# Autodesk Inventor assembly: Assembly
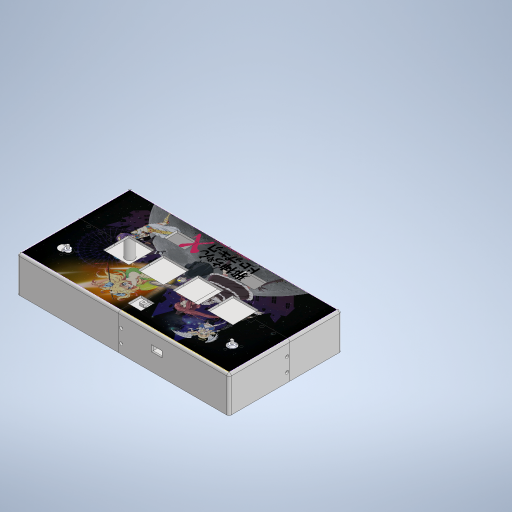
[picture p0: Inventor's stored thumbnail of the model, 512x512]
Saved by Autodesk Inventor 2023 (Build 270158000, 158)
## iProperties
Created: 2024-05-21
Part Number: Assembly
Document SubType Name: Assembly
Designer: Nitrene.P.L
Author: Nitrene.P.L
## Documents named in this file (12)
- E:\Github\AgSDVX\Hardware\Case_new\Assembly.iam
- E:\Github\AgSDVX\Hardware\Case_new\top_A.ipt
- E:\Github\AgSDVX\Hardware\Case_new\top_B.ipt
- E:\Github\AgSDVX\Hardware\Case_new\top_C.ipt
- E:\Github\AgSDVX\Hardware\Case_new\top_D.ipt
- E:\Github\AgSDVX\Hardware\Case\rotary_encoder.ipt
- E:\Github\AgSDVX\Hardware\Case_new\底板_A.ipt
- E:\Github\AgSDVX\Hardware\Case_new\底板_B.ipt
- E:\Github\AgSDVX\Hardware\Case_new\底板_C.ipt
- E:\Github\AgSDVX\Hardware\Case_new\底板_D.ipt
- E:\Github\AgSDVX\Hardware\Case_new\connect.ipt
- E:\Github\AgSDVX\Hardware\Case_new\adder.ipt
## Components (16 placed, 11 different names)
1. top_A:1 — 表面齐平:1, 配合:1, 配合:2, 表面齐平:2, 配合:3, 表面齐平:3, 插入:1, 表面齐平:7, 配合:4, 配合:5, 插入:3
2. top_B:1 — 表面齐平:1, 配合:1, 配合:2, 表面齐平:5, 插入:2, 表面齐平:8, 配合:6, 配合:7, 插入:4
3. top_C:1 — 表面齐平:2, 配合:3, 表面齐平:3, 表面齐平:4, 表面齐平:6, 表面齐平:9, 表面齐平:10, 配合:10, 配合:11
4. top_D:1 — 表面齐平:4, 表面齐平:5, 表面齐平:6, 配合:8, 配合:9
5. rotary_encoder:1 — 插入:1
6. rotary_encoder:2 — 插入:2
7. 底板_A:1 — 表面齐平:8, 配合:6, 配合:7
8. 底板_B:1 — 表面齐平:7, 配合:4, 配合:5
9. 底板_C:1 — 表面齐平:9, 配合:8, 配合:9, 配合:12, 配合:13
10. 底板_D:1 — 表面齐平:10, 配合:10, 配合:11, 配合:14, 配合:15
11. connect:1 — 配合:12
12. connect:2 — 配合:13
13. connect:3 — 配合:14
14. connect:4 — 配合:15
15. adder:1 — 插入:4
16. adder:2 — 插入:3
## Relationships (29: Mate 15, Flush 10, Insert 4)
- 表面齐平:1 [Flush]: top_A:1 ↔ top_B:1
- 配合:1 [Mate]: top_A:1 ↔ top_B:1
- 配合:2 [Mate]: top_A:1 ↔ top_B:1
- 表面齐平:2 [Flush]: top_A:1 ↔ top_C:1
- 配合:3 [Mate]: top_A:1 ↔ top_C:1
- 表面齐平:3 [Flush]: top_A:1 ↔ top_C:1
- 表面齐平:4 [Flush]: top_C:1 ↔ top_D:1
- 表面齐平:5 [Flush]: top_B:1 ↔ top_D:1
- 表面齐平:6 [Flush]: top_C:1 ↔ top_D:1
- 插入:1 [Insert]: top_A:1 ↔ rotary_encoder:1
- 插入:2 [Insert]: top_B:1 ↔ rotary_encoder:2
- 表面齐平:7 [Flush]: top_A:1 ↔ 底板_B:1
- 配合:4 [Mate]: top_A:1 ↔ 底板_B:1
- 配合:5 [Mate]: top_A:1 ↔ 底板_B:1
- 表面齐平:8 [Flush]: top_B:1 ↔ 底板_A:1
- 配合:6 [Mate]: top_B:1 ↔ 底板_A:1
- 配合:7 [Mate]: top_B:1 ↔ 底板_A:1
- 表面齐平:9 [Flush]: top_C:1 ↔ 底板_C:1
- 配合:8 [Mate]: top_D:1 ↔ 底板_C:1
- 配合:9 [Mate]: top_D:1 ↔ 底板_C:1
- 表面齐平:10 [Flush]: top_C:1 ↔ 底板_D:1
- 配合:10 [Mate]: top_C:1 ↔ 底板_D:1
- 配合:11 [Mate]: top_C:1 ↔ 底板_D:1
- 配合:12 [Mate]: 底板_C:1 ↔ connect:1
- 配合:13 [Mate]: 底板_C:1 ↔ connect:2
- 配合:14 [Mate]: 底板_D:1 ↔ connect:3
- 配合:15 [Mate]: 底板_D:1 ↔ connect:4
- 插入:3 [Insert] (-4 mm): top_A:1 ↔ adder:2
- 插入:4 [Insert] (-3 mm): top_B:1 ↔ adder:1
